# Autodesk Inventor assembly: 1_link
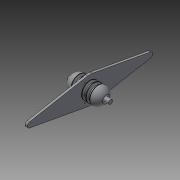
[picture p0: Inventor's stored thumbnail of the model, 180x180]
Saved by Autodesk Inventor 2014 SP1 (Build 180222100, 222)
## iProperties
Created: 2014-11-10
Part Number: 1_link
Document SubType Name: Assembly
Designer: rawrdong
Author: rawrdong
## Documents named in this file (3)
- C:\Users\rawrdong\Documents\GitHub\FlippityFlappity\CAD_HW\1_link.iam
- C:\Users\rawrdong\Documents\GitHub\FlippityFlappity\CAD_HW\VertebraeSimple.ipt
- C:\Users\rawrdong\Documents\GitHub\FlippityFlappity\CAD_HW\RibSimple.ipt
## Components (3 placed, 2 different names)
1. RibSimple:1 — Mate:1, Mate:2, Mate:3, Mate:4
2. VertebraeSimple:1 — Mate:3, Mate:4
3. VertebraeSimple:2 — Mate:1, Mate:2
## Relationships (4: Mate 4)
- Mate:1: RibSimple:1 ↔ VertebraeSimple:2
- Mate:2: RibSimple:1 ↔ VertebraeSimple:2
- Mate:3: RibSimple:1 ↔ VertebraeSimple:1
- Mate:4: RibSimple:1 ↔ VertebraeSimple:1
